# Autodesk Inventor assembly: ARM Real
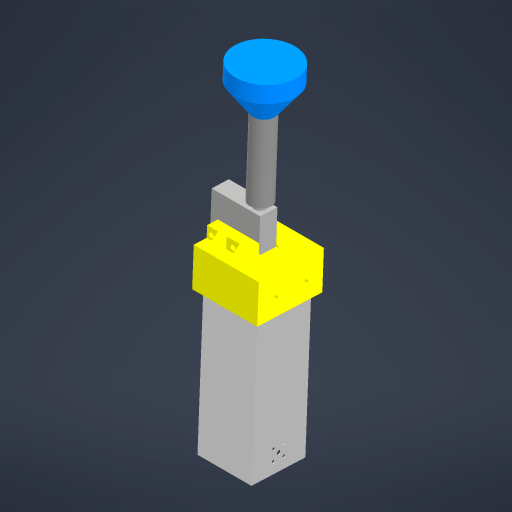
[picture p0: Inventor's stored thumbnail of the model, 512x512]
Saved by Autodesk Inventor 2023 (Build 270158000, 158)
## iProperties
Created: 2023-08-13
Part Number: ARM Real
Document SubType Name: Assembly
Designer: Abhinav
Author: Abhinav
## Documents named in this file (4)
- C:\Users\Abhinav\Desktop\GRID\ARM 3\End-Effector\00_End-Effector.iam
- C:\Users\Abhinav\Desktop\GRID\ARM 3\End-Effector\End-Link.ipt
- C:\Users\Abhinav\Desktop\GRID\ARM 3\End-Effector\Suction.ipt
- C:\Users\Abhinav\Desktop\GRID\ARM 3\End-Effector\Suction-brack.ipt
## Components (3 placed, 3 different names)
1. End-Link:1 — Mate:29, Mate:30, Mate:31
2. Suction:1 — Mate:32, Mate:33, Mate:34
3. Suction-brack:1 — Mate:29, Mate:30, Mate:31, Mate:32, Mate:33, Mate:34
## Relationships (6: Mate 6)
- Mate:29: End-Link:1 ↔ Suction-brack:1
- Mate:30: End-Link:1 ↔ Suction-brack:1
- Mate:31 (0.15 mm): End-Link:1 ↔ Suction-brack:1
- Mate:32: Suction:1 ↔ Suction-brack:1
- Mate:33: Suction:1 ↔ Suction-brack:1
- Mate:34 (0.15 mm): Suction:1 ↔ Suction-brack:1
